# Autodesk Inventor assembly: 組合3-5
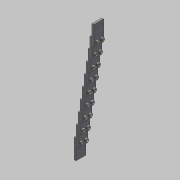
[picture p0: Inventor's stored thumbnail of the model, 180x180]
Saved by Autodesk Inventor 2018 (Build 220112000, 112)
## iProperties
Created: 2020-09-23
Part Number: 組合3-5
Material: 一般
Document SubType Name: Assembly
Designer: 王鼎鈞
Author: 王鼎鈞
## Documents named in this file (4)
- D:\2020嚴家明 功課黨\組合3-5.iam
- D:\2020嚴家明 功課黨\exercise3-3.ipt
- D:\2020嚴家明 功課黨\exercise3-4.ipt
- D:\2020嚴家明 功課黨\CNS 3932 - M 10 x 1.25 x 20-3-5螺絲.ipt
## Components (28 placed, 3 different names)
1. exercise3-3:1 — 貼合:1, 貼合:2, 貼合:3, 插入:1, 插入:2, 插入:3, 貼合:4
2. exercise3-4:1 — 貼合:1, 貼合:2, 貼合:3
3. CNS 3932 - M 10 x 1.25 x 20-3-5螺絲:1 — 插入:1
4. CNS 3932 - M 10 x 1.25 x 20-3-5螺絲:2 — 插入:2
5. exercise3-3:2 — 插入:3, 貼合:4, 插入:4, 插入:5, 插入:6, 貼合:5
6. exercise3-3:3 — 插入:18, 貼合:9, 插入:19, 插入:20, 插入:21, 貼合:10
7. exercise3-3:4 — 插入:12, 貼合:7, 插入:13, 插入:14, 插入:15, 貼合:8
8. exercise3-3:5 — 插入:21, 貼合:10, 插入:22, 插入:23, 插入:24, 貼合:11
9. exercise3-3:6 — 插入:24, 貼合:11, 插入:25, 插入:26
10. exercise3-3:7 — 插入:6, 貼合:5, 插入:7, 插入:8, 插入:9, 貼合:6
11. exercise3-3:8 — 插入:15, 貼合:8, 插入:16, 插入:17, 插入:18, 貼合:9
12. exercise3-3:9 — 插入:9, 貼合:6, 插入:10, 插入:11, 插入:12, 貼合:7
13. CNS 3932 - M 10 x 1.25 x 20-3-5螺絲:3 — 插入:4
14. CNS 3932 - M 10 x 1.25 x 20-3-5螺絲:4 — 插入:5
15. CNS 3932 - M 10 x 1.25 x 20-3-5螺絲:5 — 插入:8
16. CNS 3932 - M 10 x 1.25 x 20-3-5螺絲:6 — 插入:7
17. CNS 3932 - M 10 x 1.25 x 20-3-5螺絲:7 — 插入:11
18. CNS 3932 - M 10 x 1.25 x 20-3-5螺絲:8 — 插入:10
19. CNS 3932 - M 10 x 1.25 x 20-3-5螺絲:9 — 插入:13
20. CNS 3932 - M 10 x 1.25 x 20-3-5螺絲:10 — 插入:14
21. CNS 3932 - M 10 x 1.25 x 20-3-5螺絲:11 — 插入:17
22. CNS 3932 - M 10 x 1.25 x 20-3-5螺絲:12 — 插入:16
23. CNS 3932 - M 10 x 1.25 x 20-3-5螺絲:13 — 插入:19
24. CNS 3932 - M 10 x 1.25 x 20-3-5螺絲:14 — 插入:20
25. CNS 3932 - M 10 x 1.25 x 20-3-5螺絲:15 — 插入:22
26. CNS 3932 - M 10 x 1.25 x 20-3-5螺絲:16 — 插入:23
27. CNS 3932 - M 10 x 1.25 x 20-3-5螺絲:17 — 插入:26
28. CNS 3932 - M 10 x 1.25 x 20-3-5螺絲:18 — 插入:25
## Relationships (37: Insert 26, Mate 11)
- 貼合:1 [Mate]: exercise3-3:1 ↔ exercise3-4:1
- 貼合:2 [Mate]: exercise3-3:1 ↔ exercise3-4:1
- 貼合:3 [Mate]: exercise3-3:1 ↔ exercise3-4:1
- 插入:1 [Insert]: exercise3-3:1 ↔ CNS 3932 - M 10 x 1.25 x 20-3-5螺絲:1
- 插入:2 [Insert]: exercise3-3:1 ↔ CNS 3932 - M 10 x 1.25 x 20-3-5螺絲:2
- 插入:3 [Insert]: exercise3-3:1 ↔ exercise3-3:2
- 貼合:4 [Mate]: exercise3-3:1 ↔ exercise3-3:2
- 插入:4 [Insert]: exercise3-3:2 ↔ CNS 3932 - M 10 x 1.25 x 20-3-5螺絲:3
- 插入:5 [Insert]: exercise3-3:2 ↔ CNS 3932 - M 10 x 1.25 x 20-3-5螺絲:4
- 插入:6 [Insert]: exercise3-3:2 ↔ exercise3-3:7
- 貼合:5 [Mate]: exercise3-3:2 ↔ exercise3-3:7
- 插入:7 [Insert]: exercise3-3:7 ↔ CNS 3932 - M 10 x 1.25 x 20-3-5螺絲:6
- 插入:8 [Insert]: exercise3-3:7 ↔ CNS 3932 - M 10 x 1.25 x 20-3-5螺絲:5
- 插入:9 [Insert]: exercise3-3:7 ↔ exercise3-3:9
- 貼合:6 [Mate]: exercise3-3:7 ↔ exercise3-3:9
- 插入:10 [Insert]: exercise3-3:9 ↔ CNS 3932 - M 10 x 1.25 x 20-3-5螺絲:8
- 插入:11 [Insert]: exercise3-3:9 ↔ CNS 3932 - M 10 x 1.25 x 20-3-5螺絲:7
- 插入:12 [Insert]: exercise3-3:4 ↔ exercise3-3:9
- 貼合:7 [Mate]: exercise3-3:4 ↔ exercise3-3:9
- 插入:13 [Insert]: exercise3-3:4 ↔ CNS 3932 - M 10 x 1.25 x 20-3-5螺絲:9
- 插入:14 [Insert]: exercise3-3:4 ↔ CNS 3932 - M 10 x 1.25 x 20-3-5螺絲:10
- 插入:15 [Insert]: exercise3-3:4 ↔ exercise3-3:8
- 貼合:8 [Mate]: exercise3-3:4 ↔ exercise3-3:8
- 插入:16 [Insert]: exercise3-3:8 ↔ CNS 3932 - M 10 x 1.25 x 20-3-5螺絲:12
- 插入:17 [Insert]: exercise3-3:8 ↔ CNS 3932 - M 10 x 1.25 x 20-3-5螺絲:11
- 插入:18 [Insert]: exercise3-3:3 ↔ exercise3-3:8
- 貼合:9 [Mate]: exercise3-3:3 ↔ exercise3-3:8
- 插入:19 [Insert]: exercise3-3:3 ↔ CNS 3932 - M 10 x 1.25 x 20-3-5螺絲:13
- 插入:20 [Insert]: exercise3-3:3 ↔ CNS 3932 - M 10 x 1.25 x 20-3-5螺絲:14
- 插入:21 [Insert]: exercise3-3:3 ↔ exercise3-3:5
- 貼合:10 [Mate]: exercise3-3:3 ↔ exercise3-3:5
- 插入:22 [Insert]: exercise3-3:5 ↔ CNS 3932 - M 10 x 1.25 x 20-3-5螺絲:15
- 插入:23 [Insert]: exercise3-3:5 ↔ CNS 3932 - M 10 x 1.25 x 20-3-5螺絲:16
- 插入:24 [Insert]: exercise3-3:5 ↔ exercise3-3:6
- 貼合:11 [Mate]: exercise3-3:5 ↔ exercise3-3:6
- 插入:25 [Insert]: exercise3-3:6 ↔ CNS 3932 - M 10 x 1.25 x 20-3-5螺絲:18
- 插入:26 [Insert]: exercise3-3:6 ↔ CNS 3932 - M 10 x 1.25 x 20-3-5螺絲:17
